# Autodesk Inventor assembly: BeltDriveTest
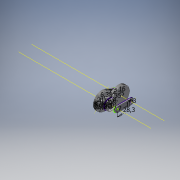
[picture p0: Inventor's stored thumbnail of the model, 180x180]
Saved by Autodesk Inventor 2018.3 (Build 223284000, 284)
## iProperties
Created: 2018-07-29
Part Number: BeltDriveTest
Material: Generisch
Document SubType Name: Assembly
Designer: JochenAlt
Author: JochenAlt
## Documents named in this file (5)
- D:\Projects\FlowerPot\CAD\Beltdrive\BeltDriveTestBed.iam
- D:\Projects\FlowerPot\CAD\Beltdrive\BeltDriveConstruction.iam
- D:\Projects\FlowerPot\CAD\Beltdrive\BeltDriveTestHolder.ipt
- D:\Projects\FlowerPot\CAD\Mounting Hub.ipt
- D:\Projects\FlowerPot\CAD\Beltdrive\ZwischenScheiben.ipt
## Components (5 placed, 4 different names)
1. BeltDriveConstruction:1 [sub-assembly] — Passend:1, Passend:2, Passend:3, Passend:5, Passend:6, Passend:13, Passend:15, Fluchtend:1, Drehung:1, Drehung:2, Passend:16
2. BeltDriveTestHolder:1 — Passend:3, Passend:9, Passend:12
3. BeltDriveTestHolder:2 — Passend:1, Passend:2, Passend:12
4. Mounting Hub:1 — Passend:5, Passend:6, Passend:9
5. Synchrone Riemenscheibe1:1 — Passend:13, Drehung:1, Drehung:2
## Relationships (13: Mate 10, RelateRotation 2, Flush 1)
- Passend:1 [Mate]: BeltDriveConstruction:1 ↔ BeltDriveTestHolder:2
- Passend:2 [Mate] (0.04 mm): BeltDriveConstruction:1 ↔ BeltDriveTestHolder:2
- Passend:3 [Mate]: BeltDriveConstruction:1 ↔ BeltDriveTestHolder:1
- Passend:5 [Mate]: BeltDriveConstruction:1 ↔ Mounting Hub:1
- Passend:6 [Mate]: BeltDriveConstruction:1 ↔ Mounting Hub:1
- Passend:9 [Mate] (1 mm): BeltDriveTestHolder:1 ↔ Mounting Hub:1
- Passend:12 [Mate]: BeltDriveTestHolder:1 ↔ BeltDriveTestHolder:2
- Passend:13 [Mate]: BeltDriveConstruction:1 ↔ Synchrone Riemenscheibe1:1
- Passend:15 [Mate]: BeltDriveConstruction:1
- Fluchtend:1 [Flush]: BeltDriveConstruction:1
- Drehung:1 [RelateRotation] (3 ul): BeltDriveConstruction:1 ↔ Synchrone Riemenscheibe1:1
- Drehung:2 [RelateRotation] (0.3333 ul): BeltDriveConstruction:1 ↔ Synchrone Riemenscheibe1:1
- Passend:16 [Mate]: BeltDriveConstruction:1
